# Autodesk Inventor assembly: Hotend 2.2
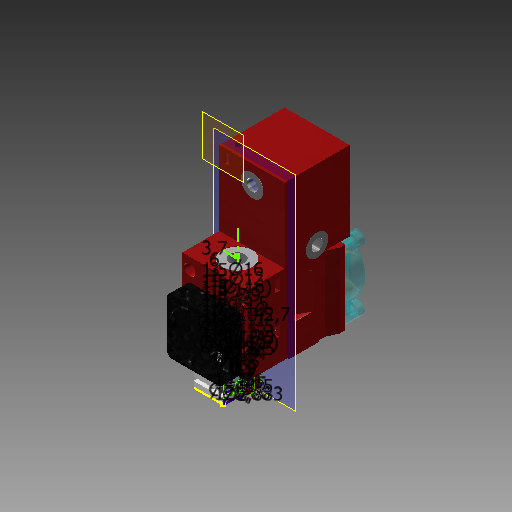
[picture p0: Inventor's stored thumbnail of the model, 512x512]
Saved by Autodesk Inventor 2018.1 (Build 221171000, 171)
## iProperties
Part Number: Hotend 2.2
Material: Generisch
Document SubType Name: Assembly
Designer: Till
Author: Till
## Documents named in this file (7)
- C:\Users\tillm\Dropbox\Ultibox\ultibox\cad\Hotend 2.2.iam
- C:\Users\tillm\Dropbox\Ultibox\ultibox\cad\Hotend Mount 2.2.ipt
- C:\Users\tillm\Dropbox\Ultibox\ultibox\cad\E3D-HotEnd.iam
- C:\Users\tillm\Dropbox\Ultibox\ultibox\cad\Clamp.ipt
- C:\Users\tillm\Dropbox\Ultibox\ultibox\cad\LM6LUU.ipt
- C:\Users\tillm\Dropbox\Ultibox\ultibox\cad\CPU - -KF0410-01.ipt
- C:\Users\tillm\Dropbox\Ultibox\ultibox\cad\30mm Fan.ipt
## Components (7 placed, 6 different names)
1. Hotend Mount 2.2:1 — Passend:1, Passend:2, Fluchtend:1, Passend:3, Fluchtend:2, Fluchtend:3, Fluchtend:4, Fluchtend:5, Passend:6, Passend:7, Fluchtend:7, Fluchtend:8, Passend:11, Passend:12, Passend:13
2. E3D-HotEnd:1 [sub-assembly] — Passend:3, Fluchtend:2
3. Clamp:1 — Fluchtend:3, Fluchtend:4, Fluchtend:5, Passend:8, Passend:9, Passend:10
4. LM6LUU:1 — Passend:7, Fluchtend:7
5. LM6LUU:2 — Passend:6, Fluchtend:8
6. CPU - -KF0410-01:1 — Passend:11, Passend:12, Passend:13
7. 30mm Fan:1 — Passend:8, Passend:9, Passend:10
## Relationships (18: Mate 11, Flush 7)
- Passend:1 [Mate]: Hotend Mount 2.2:1
- Passend:2 [Mate]: Hotend Mount 2.2:1
- Fluchtend:1 [Flush]: Hotend Mount 2.2:1
- Passend:3 [Mate]: Hotend Mount 2.2:1 ↔ E3D-HotEnd:1
- Fluchtend:2 [Flush]: Hotend Mount 2.2:1 ↔ E3D-HotEnd:1
- Fluchtend:3 [Flush]: Hotend Mount 2.2:1 ↔ Clamp:1
- Fluchtend:4 [Flush]: Hotend Mount 2.2:1 ↔ Clamp:1
- Fluchtend:5 [Flush]: Hotend Mount 2.2:1 ↔ Clamp:1
- Passend:6 [Mate]: Hotend Mount 2.2:1 ↔ LM6LUU:2
- Passend:7 [Mate]: Hotend Mount 2.2:1 ↔ LM6LUU:1
- Fluchtend:7 [Flush]: Hotend Mount 2.2:1 ↔ LM6LUU:1
- Fluchtend:8 [Flush]: Hotend Mount 2.2:1 ↔ LM6LUU:2
- Passend:8 [Mate]: Clamp:1 ↔ 30mm Fan:1
- Passend:9 [Mate]: Clamp:1 ↔ 30mm Fan:1
- Passend:10 [Mate]: Clamp:1 ↔ 30mm Fan:1
- Passend:11 [Mate]: Hotend Mount 2.2:1 ↔ CPU - -KF0410-01:1
- Passend:12 [Mate]: Hotend Mount 2.2:1 ↔ CPU - -KF0410-01:1
- Passend:13 [Mate]: Hotend Mount 2.2:1 ↔ CPU - -KF0410-01:1
